# Autodesk Inventor assembly: LPC
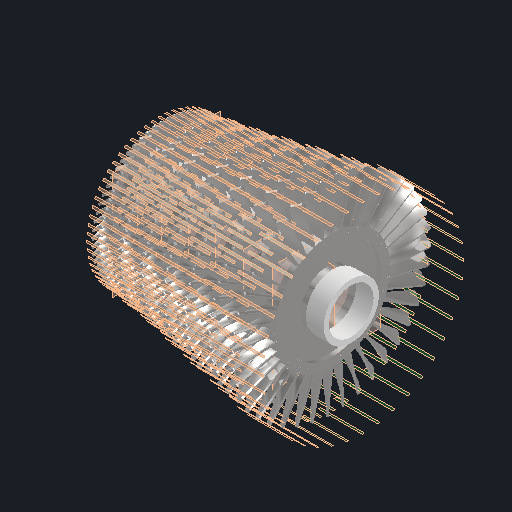
[picture p0: Inventor's stored thumbnail of the model, 512x512]
Saved by Autodesk Inventor 2026.2 (Build 302298010, 298A)
## iProperties
Created: 2026-04-26
Part Number: LPC
Document SubType Name: Assembly
Designer: Yan
Author: Yan
## Documents named in this file (12)
- C:\Users\Yan\Desktop\Turbina\LPC.iam
- C:\Users\Yan\Desktop\Turbina\Stadio5.iam
- C:\Users\Yan\Desktop\Turbina\Stadio6.iam
- C:\Users\Yan\Desktop\Turbina\Stadio7.iam
- C:\Users\Yan\Desktop\Turbina\Stadio8.iam
- C:\Users\Yan\Desktop\Turbina\Stadio9.iam
- C:\Users\Yan\Desktop\Turbina\Stadio10.iam
- C:\Users\Yan\Desktop\Turbina\Stadio4.iam
- C:\Users\Yan\Desktop\Turbina\Spaziamento4-5-6ipt.ipt
- C:\Users\Yan\Desktop\Turbina\Spaziamento6-7-8ipt.ipt
- C:\Users\Yan\Desktop\Turbina\Spaziamento8-9-10ipt.ipt
- C:\Users\Yan\Desktop\Turbina\Spaziamento3-4ipt.ipt
## Components (15 placed, 11 different names)
1. Stadio5:1 [sub-assembly] — Mate:3, Mate:4, Mate:5, Mate:10
2. Stadio6:1 [sub-assembly] — Mate:7, Mate:8, Mate:9, Mate:16
3. Stadio7:1 [sub-assembly] — Mate:11, Mate:12, Mate:13, Mate:14, Mate:18
4. Stadio8:1 [sub-assembly] — Mate:15, Mate:16, Mate:17
5. Stadio9:1 [sub-assembly] — Mate:19, Mate:20, Mate:21, Mate:22, Mate:24
6. Stadio10:1 [sub-assembly] — Mate:23, Mate:24, Mate:25, Mate:26
7. Stadio4:1 [sub-assembly] — Mate:1, Mate:2, Mate:4, Mate:6, Mate:27, Mate:28
8. Spaziamento4-5-6ipt:1 — Mate:1, Mate:2, Mate:3
9. Spaziamento4-5-6ipt:2 — Mate:5, Mate:6, Mate:7, Mate:8
10. Spaziamento6-7-8ipt:1 — Mate:9, Mate:10, Mate:11, Mate:12, Mate:20
11. Spaziamento6-7-8ipt:2 — Mate:13, Mate:14, Mate:15
12. Spaziamento8-9-10ipt:1 — Mate:17, Mate:18, Mate:19
13. Spaziamento8-9-10ipt:2 — Mate:21, Mate:22, Mate:23
14. Spaziamento3-4ipt:1 — Mate:27, Mate:28
15. Spaziamento8-9-10ipt:3 — Mate:25, Mate:26
## Relationships (28: Mate 28)
- Mate:1: Stadio4:1 ↔ Spaziamento4-5-6ipt:1
- Mate:2: Stadio4:1 ↔ Spaziamento4-5-6ipt:1
- Mate:3: Stadio5:1 ↔ Spaziamento4-5-6ipt:1
- Mate:4: Stadio5:1 ↔ Stadio4:1
- Mate:5: Stadio5:1 ↔ Spaziamento4-5-6ipt:2
- Mate:6: Stadio4:1 ↔ Spaziamento4-5-6ipt:2
- Mate:7: Stadio6:1 ↔ Spaziamento4-5-6ipt:2
- Mate:8: Stadio6:1 ↔ Spaziamento4-5-6ipt:2
- Mate:9: Stadio6:1 ↔ Spaziamento6-7-8ipt:1
- Mate:10: Stadio5:1 ↔ Spaziamento6-7-8ipt:1
- Mate:11: Stadio7:1 ↔ Spaziamento6-7-8ipt:1
- Mate:12: Stadio7:1 ↔ Spaziamento6-7-8ipt:1
- Mate:13: Stadio7:1 ↔ Spaziamento6-7-8ipt:2
- Mate:14: Stadio7:1 ↔ Spaziamento6-7-8ipt:2
- Mate:15: Stadio8:1 ↔ Spaziamento6-7-8ipt:2
- Mate:16: Stadio6:1 ↔ Stadio8:1
- Mate:17: Stadio8:1 ↔ Spaziamento8-9-10ipt:1
- Mate:18: Stadio7:1 ↔ Spaziamento8-9-10ipt:1
- Mate:19: Stadio9:1 ↔ Spaziamento8-9-10ipt:1
- Mate:20: Stadio9:1 ↔ Spaziamento6-7-8ipt:1
- Mate:21: Stadio9:1 ↔ Spaziamento8-9-10ipt:2
- Mate:22: Stadio9:1 ↔ Spaziamento8-9-10ipt:2
- Mate:23: Stadio10:1 ↔ Spaziamento8-9-10ipt:2
- Mate:24: Stadio9:1 ↔ Stadio10:1
- Mate:25: Stadio10:1 ↔ Spaziamento8-9-10ipt:3
- Mate:26: Stadio10:1 ↔ Spaziamento8-9-10ipt:3
- Mate:27: Stadio4:1 ↔ Spaziamento3-4ipt:1
- Mate:28: Stadio4:1 ↔ Spaziamento3-4ipt:1
